# Autodesk Inventor assembly: Selection_Shaft Assy
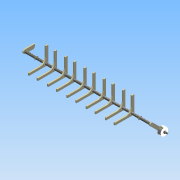
[picture p0: Inventor's stored thumbnail of the model, 180x180]
Saved by Autodesk Inventor 2018.1 (Build 221171000, 171)
## iProperties
Created: 2019-02-14
Part Number: Selection_Shaft Assy
Document SubType Name: Assembly
Designer: James
Author: James
## Documents named in this file (9)
- C:\Users\admin\Desktop\Ball Sorting Machine\Ball-Sorting-Machine\Prototype CAD\Selection Sort - 40mm\Prototype_Shaft Assy.iam
- C:\Users\admin\Desktop\Ball Sorting Machine\Ball-Sorting-Machine\Prototype CAD\Selection Sort - 40mm\Prototype_Shaft 1.ipt
- C:\Users\admin\Desktop\Ball Sorting Machine\Ball-Sorting-Machine\Prototype CAD\Selection Sort - 40mm\Prototype_Selector 1.ipt
- C:\Users\admin\Desktop\Ball Sorting Machine\Ball-Sorting-Machine\Prototype CAD\Selection Sort - 40mm\BS 3673 - 6mm External Circlip.ipt
- C:\Users\admin\Desktop\Ball Sorting Machine\Ball-Sorting-Machine\Prototype CAD\Selection Sort - 40mm\Prototype_Counterweight.ipt
- C:\Users\admin\Desktop\Ball Sorting Machine\Ball-Sorting-Machine\Prototype CAD\Selection Sort - 40mm\M3 x 20 - Hex. Head Set Screw (MS).ipt
- C:\Users\admin\Desktop\Ball Sorting Machine\Ball-Sorting-Machine\Prototype CAD\Selection Sort - 40mm\Locknut - M3.ipt
- C:\Users\admin\Desktop\Ball Sorting Machine\Ball-Sorting-Machine\Prototype CAD\Selection Sort - 40mm\Prototype_Weight.ipt
- C:\Users\admin\Desktop\Ball Sorting Machine\Ball-Sorting-Machine\Prototype CAD\Selection Sort - 40mm\Prototype_Lever 2.ipt
## Components (31 placed, 8 different names)
1. Prototype_Shaft 1:1 — Flush:1, Flush:2, Flush:3, Mate:1, Mate:2, Flush:5, Flush:6, Mate:3, Mate:4, Mate:5, Mate:6, Mate:7, Mate:8, Mate:9, Mate:10, Mate:11, Mate:12, Mate:25, Mate:26
2. BS 3673 - 6mm External Circlip:11 — Mate:7, Mate:8, Flush:8
3. BS 3673 - 6mm External Circlip:12 — Mate:9, Mate:10, Flush:7, Flush:8
4. Prototype_Counterweight:1 — Mate:11, Angle:1, Mate:12, Mate:13, Mate:14, Mate:17
5. Hex. Head Set Screw (MS) - M3 x 10:1 — Mate:13, Mate:14, Mate:15, Mate:16, Mate:22, Mate:23, Mate:24
6. Locknut - M3:1 — Mate:15, Mate:21
7. Prototype_Weight:1 — Mate:16, Mate:17, Mate:18
8. Prototype_Weight:2 — Mate:18, Mate:19, Mate:24
9. Prototype_Weight:3 — Mate:19, Mate:20, Mate:23
10. Prototype_Weight:4 — Mate:20, Mate:21, Mate:22
11. Prototype_Lever 2:1 — Mate:25, Mate:26, Angle:2
12. BS 3673 - 6mm External Circlip:2 — Mate:4, Mate:5, Flush:7, Flush:9
13. Prototype_Selector 1:1 — Mate:2, Flush:4, Flush:5, Angle:1
14. BS 3673 - 6mm External Circlip:1 — Mate:3, Mate:6, Flush:9
15. Prototype_Selector 1:2 — Mate:1, Flush:4, Flush:6
16. BS 3673 - 6mm External Circlip:3
17. Prototype_Selector 1:3
18. BS 3673 - 6mm External Circlip:4
19. Prototype_Selector 1:4
20. BS 3673 - 6mm External Circlip:5
21. Prototype_Selector 1:5
22. BS 3673 - 6mm External Circlip:6
23. Prototype_Selector 1:6
24. BS 3673 - 6mm External Circlip:7
25. Prototype_Selector 1:7
26. BS 3673 - 6mm External Circlip:8
27. Prototype_Selector 1:8
28. BS 3673 - 6mm External Circlip:9
29. Prototype_Selector 1:9
30. BS 3673 - 6mm External Circlip:10
31. Prototype_Selector 1:10 — Angle:2
## Component patterns: (5 elements, first: BS 3673 - 6mm External Circlip:2 + Prototype_Selector 1:1 + BS 3673 - 6mm External Circlip:1 + Prototype_Selector 1:2)
## Relationships (37: Mate 26, Flush 9, Angle 2)
- Flush:1: Prototype_Shaft 1:1
- Flush:2: Prototype_Shaft 1:1
- Flush:3: Prototype_Shaft 1:1
- Mate:1: Prototype_Shaft 1:1 ↔ Prototype_Selector 1:2
- Mate:2: Prototype_Shaft 1:1 ↔ Prototype_Selector 1:1
- Flush:4: Prototype_Selector 1:1 ↔ Prototype_Selector 1:2
- Flush:5: Prototype_Shaft 1:1 ↔ Prototype_Selector 1:1
- Flush:6: Prototype_Shaft 1:1 ↔ Prototype_Selector 1:2
- Mate:3: Prototype_Shaft 1:1 ↔ BS 3673 - 6mm External Circlip:1
- Mate:4: Prototype_Shaft 1:1 ↔ BS 3673 - 6mm External Circlip:2
- Mate:5: Prototype_Shaft 1:1 ↔ BS 3673 - 6mm External Circlip:2
- Mate:6: Prototype_Shaft 1:1 ↔ BS 3673 - 6mm External Circlip:1
- Mate:7: Prototype_Shaft 1:1 ↔ BS 3673 - 6mm External Circlip:11
- Mate:8: Prototype_Shaft 1:1 ↔ BS 3673 - 6mm External Circlip:11
- Mate:9: Prototype_Shaft 1:1 ↔ BS 3673 - 6mm External Circlip:12
- Mate:10: Prototype_Shaft 1:1 ↔ BS 3673 - 6mm External Circlip:12
- Flush:7: BS 3673 - 6mm External Circlip:12 ↔ BS 3673 - 6mm External Circlip:2
- Flush:8: BS 3673 - 6mm External Circlip:11 ↔ BS 3673 - 6mm External Circlip:12
- Mate:11: Prototype_Shaft 1:1 ↔ Prototype_Counterweight:1
- Angle:1 (45 deg): Prototype_Counterweight:1 ↔ Prototype_Selector 1:1
- Mate:12: Prototype_Shaft 1:1 ↔ Prototype_Counterweight:1
- Flush:9: BS 3673 - 6mm External Circlip:2 ↔ BS 3673 - 6mm External Circlip:1
- Mate:13: Prototype_Counterweight:1 ↔ Hex. Head Set Screw (MS) - M3 x 10:1
- Mate:14: Prototype_Counterweight:1 ↔ Hex. Head Set Screw (MS) - M3 x 10:1
- Mate:15: Hex. Head Set Screw (MS) - M3 x 10:1 ↔ Locknut - M3:1
- Mate:16: Hex. Head Set Screw (MS) - M3 x 10:1 ↔ Prototype_Weight:1
- Mate:17: Prototype_Counterweight:1 ↔ Prototype_Weight:1
- Mate:18: Prototype_Weight:1 ↔ Prototype_Weight:2
- Mate:19: Prototype_Weight:2 ↔ Prototype_Weight:3
- Mate:20: Prototype_Weight:3 ↔ Prototype_Weight:4
- Mate:21: Locknut - M3:1 ↔ Prototype_Weight:4
- Mate:22: Hex. Head Set Screw (MS) - M3 x 10:1 ↔ Prototype_Weight:4
- Mate:23: Hex. Head Set Screw (MS) - M3 x 10:1 ↔ Prototype_Weight:3
- Mate:24: Hex. Head Set Screw (MS) - M3 x 10:1 ↔ Prototype_Weight:2
- Mate:25: Prototype_Shaft 1:1 ↔ Prototype_Lever 2:1
- Mate:26: Prototype_Shaft 1:1 ↔ Prototype_Lever 2:1
- Angle:2 (0 deg): Prototype_Lever 2:1 ↔ Prototype_Selector 1:10
